# Autodesk Inventor assembly: GE-13016
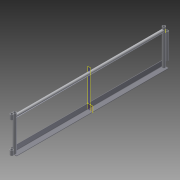
[picture p0: Inventor's stored thumbnail of the model, 180x180]
Saved by Autodesk Inventor 2013 (Build 170138000, 138)
## iProperties
Created: 2012-12-31
Part Number: GE-13016
Document SubType Name: Assembly
Designer: Phillip
Author: Phillip
## Documents named in this file (3)
- E:\Data Folder\FIRST 2013\FIRST KOP\FIRST Arena 2013\Feeder Goal Station\GE-13016.iam
- E:\Data Folder\FIRST 2013\FIRST KOP\FIRST Arena 2013\Feeder Goal Station\GE-13015-01.ipt
- E:\Data Folder\FIRST 2013\FIRST KOP\FIRST Arena 2013\Feeder Goal Station\GE-13016_Frame.iam
## Components (2 placed, 2 different names)
1. GE-13015-01:1 — Tangent:1, Tangent:2, Mate:1, Mate:2, Mate:3, Angle:1
2. GE-13016_Frame:1 [sub-assembly] — Tangent:1, Tangent:2, Mate:1, Mate:2, Flush:1
## Relationships (8: Mate 4, Tangent 2, Angle 1, Flush 1)
- Tangent:1: GE-13015-01:1 ↔ GE-13016_Frame:1
- Tangent:2: GE-13015-01:1 ↔ GE-13016_Frame:1
- Mate:1: GE-13015-01:1 ↔ GE-13016_Frame:1
- Mate:2: GE-13015-01:1 ↔ GE-13016_Frame:1
- Mate:3: GE-13015-01:1
- Angle:1 (0 deg): GE-13015-01:1
- Flush:1 (-1071.626 mm): GE-13016_Frame:1
- Mate:4
